# Autodesk Inventor assembly: Krzyżyk
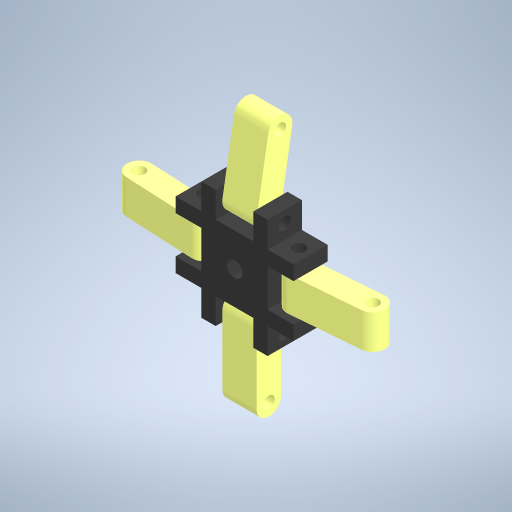
[picture p0: Inventor's stored thumbnail of the model, 512x512]
Saved by Autodesk Inventor 2023 (Build 270158000, 158)
## iProperties
Created: 2023-06-03
Part Number: Krzyżyk
Document SubType Name: Assembly
Designer: Kamil
Author: Kamil
## Documents named in this file (3)
- C:\Users\Kamil\Desktop\KONARM_2\chwytak\Krzyżyk.iam
- C:\Users\Kamil\Desktop\KONARM_2\chwytak\ArmMuscle.ipt
- C:\Users\Kamil\Desktop\KONARM_2\chwytak\GripperMotorHinges.ipt
## Components (5 placed, 2 different names)
1. ArmMuscle:1 — Równoległe:1, Zestawiające:1, Zestawiające:3
2. ArmMuscle:2 — Równoległe:1, Zestawiające:4
3. ArmMuscle:3 — Równoległe:2, Zestawiające:2, Zestawiające:5
4. ArmMuscle:4 — Równoległe:2, Zestawiające:6
5. GripperMotorHinges:1 — Zestawiające:1, Zestawiające:2, Zestawiające:3, Zestawiające:4, Zestawiające:5, Zestawiające:6
## Relationships (8: Mate 6, Flush 2)
- Równoległe:1 [Flush]: ArmMuscle:1 ↔ ArmMuscle:2
- Równoległe:2 [Flush]: ArmMuscle:3 ↔ ArmMuscle:4
- Zestawiające:1 [Mate] (0.5 mm): ArmMuscle:1 ↔ GripperMotorHinges:1
- Zestawiające:2 [Mate] (0.5 mm): ArmMuscle:3 ↔ GripperMotorHinges:1
- Zestawiające:3 [Mate]: ArmMuscle:1 ↔ GripperMotorHinges:1
- Zestawiające:4 [Mate]: ArmMuscle:2 ↔ GripperMotorHinges:1
- Zestawiające:5 [Mate]: ArmMuscle:3 ↔ GripperMotorHinges:1
- Zestawiające:6 [Mate]: ArmMuscle:4 ↔ GripperMotorHinges:1
